# Autodesk Inventor assembly: Koruza L-profil
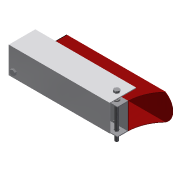
[picture p0: Inventor's stored thumbnail of the model, 180x180]
Saved by Autodesk Inventor 2015 (Build 190159000, 159)
## iProperties
Created: 2015-01-09
Part Number: Koruza L-profil
Document SubType Name: Assembly
Designer: Michal
Author: Michal
## Documents named in this file (10)
- C:\Users\Michal\Desktop\Michal\Prace\koruza\Koruza L-profil.iam
- C:\Users\Michal\Desktop\Michal\Prace\koruza\Case.ipt
- C:\Users\Michal\Desktop\Michal\Prace\koruza\U-profil 100x40 - pod case.ipt
- C:\Users\Michal\Desktop\Michal\Prace\koruza\Šrouv M12x60.ipt
- C:\Users\Michal\Desktop\Michal\Prace\koruza\ANSI B18.16.3M - Property Class 5 and 10 - Metric M12 x 1.75 Typ kovu.ipt
- C:\Users\Michal\Desktop\Michal\Prace\koruza\ISO 4035 - M12ISO.ipt
- C:\Users\Michal\Desktop\Michal\Prace\koruza\L profil 100x100 základní.ipt
- C:\Users\Michal\Desktop\Michal\Prace\koruza\Šroub M3x8.ipt
- C:\Users\Michal\Desktop\Michal\Prace\koruza\ISO 4032 - M3ISO.ipt
- C:\Users\Michal\Desktop\Michal\Prace\koruza\Zadní kryt.ipt
## Components (20 placed, 9 different names)
1. Case:1 — Proti sobě:1, Stejný směr:1, Stejný směr:2, Proti sobě:21, Proti sobě:22, Proti sobě:23, Proti sobě:24, Proti sobě:25, Proti sobě:26, Proti sobě:27, Proti sobě:28, Stejný směr:3, Stejný směr:4, Stejný směr:5
2. U-profil 100x40 - pod case:1 — Proti sobě:1, Stejný směr:1, Stejný směr:2, Proti sobě:2, Proti sobě:3, Proti sobě:4, Proti sobě:5, Proti sobě:11, Proti sobě:12, Proti sobě:16, Proti sobě:18, Proti sobě:33, Proti sobě:34, Proti sobě:35, Proti sobě:36
3. L profil 100x100 základní:1 — Proti sobě:2, Proti sobě:3, Proti sobě:4, Proti sobě:6, Proti sobě:7, Proti sobě:8, Proti sobě:14, Proti sobě:20
4. Šrouv M12x60:1 — Proti sobě:7, Proti sobě:8, Proti sobě:9, Proti sobě:10, Proti sobě:13
5. Šrouv M12x60:2 — Proti sobě:5, Proti sobě:6, Proti sobě:15, Proti sobě:17, Proti sobě:19
6. ISO 4035 - M12ISO:1 — Proti sobě:17, Proti sobě:18
7. ISO 4035 - M12ISO:2 — Proti sobě:15, Proti sobě:16
8. ISO 4035 - M12ISO:3 — Proti sobě:9, Proti sobě:11
9. ISO 4035 - M12ISO:4 — Proti sobě:10, Proti sobě:12
10. ANSI B18.16.3M - Property Class 5 and 10 - Metric M12 x 1.75 Typ kovu:1 — Proti sobě:19, Proti sobě:20
11. ANSI B18.16.3M - Property Class 5 and 10 - Metric M12 x 1.75 Typ kovu:2 — Proti sobě:13, Proti sobě:14
12. Šroub M3x8:1 — Proti sobě:25, Proti sobě:26, Proti sobě:30
13. Šroub M3x8:2 — Proti sobě:24, Proti sobě:28, Proti sobě:32
14. Šroub M3x8:3 — Proti sobě:23, Proti sobě:27, Proti sobě:31
15. Šroub M3x8:4 — Proti sobě:21, Proti sobě:22, Proti sobě:29
16. ISO 4032 - M3ISO:1 — Proti sobě:32, Proti sobě:33
17. ISO 4032 - M3ISO:2 — Proti sobě:31, Proti sobě:34
18. ISO 4032 - M3ISO:3 — Proti sobě:29, Proti sobě:36
19. ISO 4032 - M3ISO:4 — Proti sobě:30, Proti sobě:35
20. Zadní kryt:1 — Stejný směr:3, Stejný směr:4, Stejný směr:5
## Relationships (41: Mate 36, Flush 5)
- Proti sobě:1 [Mate]: Case:1 ↔ U-profil 100x40 - pod case:1
- Stejný směr:1 [Flush]: Case:1 ↔ U-profil 100x40 - pod case:1
- Stejný směr:2 [Flush] (-50 mm): Case:1 ↔ U-profil 100x40 - pod case:1
- Proti sobě:2 [Mate]: U-profil 100x40 - pod case:1 ↔ L profil 100x100 základní:1
- Proti sobě:3 [Mate] (25 mm): U-profil 100x40 - pod case:1 ↔ L profil 100x100 základní:1
- Proti sobě:4 [Mate]: U-profil 100x40 - pod case:1 ↔ L profil 100x100 základní:1
- Proti sobě:5 [Mate]: U-profil 100x40 - pod case:1 ↔ Šrouv M12x60:2
- Proti sobě:6 [Mate]: L profil 100x100 základní:1 ↔ Šrouv M12x60:2
- Proti sobě:7 [Mate]: L profil 100x100 základní:1 ↔ Šrouv M12x60:1
- Proti sobě:8 [Mate]: L profil 100x100 základní:1 ↔ Šrouv M12x60:1
- Proti sobě:9 [Mate]: Šrouv M12x60:1 ↔ ISO 4035 - M12ISO:3
- Proti sobě:10 [Mate]: Šrouv M12x60:1 ↔ ISO 4035 - M12ISO:4
- Proti sobě:11 [Mate]: U-profil 100x40 - pod case:1 ↔ ISO 4035 - M12ISO:3
- Proti sobě:12 [Mate]: U-profil 100x40 - pod case:1 ↔ ISO 4035 - M12ISO:4
- Proti sobě:13 [Mate]: Šrouv M12x60:1 ↔ ANSI B18.16.3M - Property Class 5 and 10 - Metric M12 x 1.75 Typ kovu:2
- Proti sobě:14 [Mate]: L profil 100x100 základní:1 ↔ ANSI B18.16.3M - Property Class 5 and 10 - Metric M12 x 1.75 Typ kovu:2
- Proti sobě:15 [Mate]: Šrouv M12x60:2 ↔ ISO 4035 - M12ISO:2
- Proti sobě:16 [Mate]: U-profil 100x40 - pod case:1 ↔ ISO 4035 - M12ISO:2
- Proti sobě:17 [Mate]: Šrouv M12x60:2 ↔ ISO 4035 - M12ISO:1
- Proti sobě:18 [Mate]: U-profil 100x40 - pod case:1 ↔ ISO 4035 - M12ISO:1
- Proti sobě:19 [Mate]: Šrouv M12x60:2 ↔ ANSI B18.16.3M - Property Class 5 and 10 - Metric M12 x 1.75 Typ kovu:1
- Proti sobě:20 [Mate]: L profil 100x100 základní:1 ↔ ANSI B18.16.3M - Property Class 5 and 10 - Metric M12 x 1.75 Typ kovu:1
- Proti sobě:21 [Mate]: Case:1 ↔ Šroub M3x8:4
- Proti sobě:22 [Mate]: Case:1 ↔ Šroub M3x8:4
- Proti sobě:23 [Mate]: Case:1 ↔ Šroub M3x8:3
- Proti sobě:24 [Mate]: Case:1 ↔ Šroub M3x8:2
- Proti sobě:25 [Mate]: Case:1 ↔ Šroub M3x8:1
- Proti sobě:26 [Mate]: Case:1 ↔ Šroub M3x8:1
- Proti sobě:27 [Mate]: Case:1 ↔ Šroub M3x8:3
- Proti sobě:28 [Mate]: Case:1 ↔ Šroub M3x8:2
- Proti sobě:29 [Mate]: Šroub M3x8:4 ↔ ISO 4032 - M3ISO:3
- Proti sobě:30 [Mate]: Šroub M3x8:1 ↔ ISO 4032 - M3ISO:4
- Proti sobě:31 [Mate]: Šroub M3x8:3 ↔ ISO 4032 - M3ISO:2
- Proti sobě:32 [Mate]: Šroub M3x8:2 ↔ ISO 4032 - M3ISO:1
- Proti sobě:33 [Mate]: U-profil 100x40 - pod case:1 ↔ ISO 4032 - M3ISO:1
- Proti sobě:34 [Mate]: U-profil 100x40 - pod case:1 ↔ ISO 4032 - M3ISO:2
- Proti sobě:35 [Mate]: U-profil 100x40 - pod case:1 ↔ ISO 4032 - M3ISO:4
- Proti sobě:36 [Mate]: U-profil 100x40 - pod case:1 ↔ ISO 4032 - M3ISO:3
- Stejný směr:3 [Flush]: Case:1 ↔ Zadní kryt:1
- Stejný směr:4 [Flush]: Case:1 ↔ Zadní kryt:1
- Stejný směr:5 [Flush] (-2 mm): Case:1 ↔ Zadní kryt:1
